# Autodesk Inventor assembly: Right One Motor Gearbox
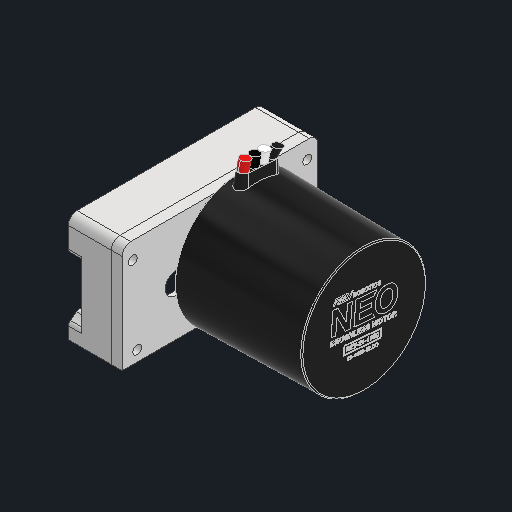
[picture p0: Inventor's stored thumbnail of the model, 512x512]
Saved by Autodesk Inventor 2022 (Build 260153000, 153)
## iProperties
Created: 2022-09-11
Part Number: Right One Motor Gearbox
Document SubType Name: Assembly
Designer: robpl
Author: robpl
## Documents named in this file (4)
- C:\Users\robpl\OneDrive\Documents\Inventor\2022 FRC Season\Best Coast Drive\Right One Motor Gearbox.iam
- C:\Users\robpl\OneDrive\Documents\Inventor\2022 FRC Season\Best Coast Drive\Right One Motor Gearbox Cover.ipt
- C:\Users\robpl\OneDrive\Documents\Inventor\2022 FRC Season\Best Coast Drive\Right One Motor Plate.ipt
- C:\Users\robpl\OneDrive\Documents\Inventor\2022 FRC Season\Best Coast Drive\NEO.ipt
## Components (3 placed, 3 different names)
1. Right One Motor Gearbox Cover:1 — Mate:1, Mate:2, Mate:3
2. Right One Motor Plate:1 — Mate:1, Mate:2, Mate:3, Mate:4, Mate:5, Mate:6
3. NEO:1 — Mate:4, Mate:5, Mate:6
## Relationships (6: Mate 6)
- Mate:1: Right One Motor Gearbox Cover:1 ↔ Right One Motor Plate:1
- Mate:2: Right One Motor Gearbox Cover:1 ↔ Right One Motor Plate:1
- Mate:3: Right One Motor Gearbox Cover:1 ↔ Right One Motor Plate:1
- Mate:4: Right One Motor Plate:1 ↔ NEO:1
- Mate:5: Right One Motor Plate:1 ↔ NEO:1
- Mate:6: Right One Motor Plate:1 ↔ NEO:1
